# Autodesk Inventor assembly: bear_89_140
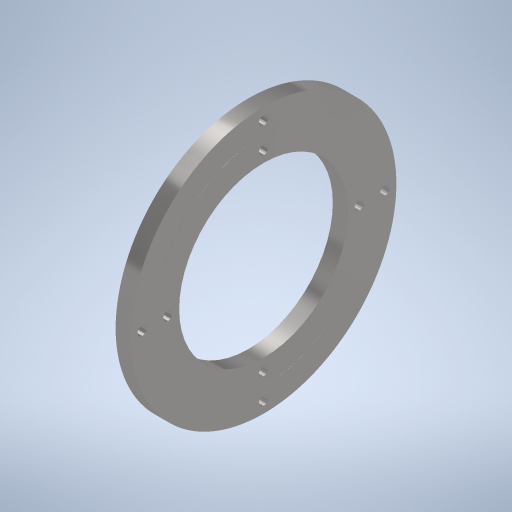
[picture p0: Inventor's stored thumbnail of the model, 512x512]
Saved by Autodesk Inventor 2024.1 (Build 281209000, 209)
## iProperties
Created: 2023-06-29
Part Number: bear_89_140
Document SubType Name: Assembly
Designer: fhbdh
Author: fhbdh
## Documents named in this file (3)
- C:\Users\haruy\OneDrive - Kyushu University\KURT_工房共有\2023~2024\ハード\CAD\2024NHK\000_parts\回転台\bear_89_140.iam
- C:\Users\haruy\OneDrive - Kyushu University\KURT_工房共有\2023~2024\ハード\CAD\2024NHK\nagahisa\normal_ver2.0-takagicopy\frequently used parts\ベアリング\bear_89_140\bear_89_140_in.ipt
- C:\Users\haruy\OneDrive - Kyushu University\KURT_工房共有\2023~2024\ハード\CAD\2024NHK\nagahisa\normal_ver2.0-takagicopy\frequently used parts\ベアリング\bear_89_140\bear_89_140_out.ipt
## Components (2 placed, 2 different names)
1. bear_89_140_in:1 — 挿入:1
2. bear_89_140_out:1 — 挿入:1
## Relationships (1: Insert 1)
- 挿入:1 [Insert]: bear_89_140_in:1 ↔ bear_89_140_out:1
